# Autodesk Inventor assembly: front
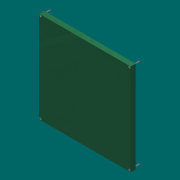
[picture p0: Inventor's stored thumbnail of the model, 180x180]
Saved by Autodesk Inventor 2016 (Build 200138000, 138)
## iProperties
Created: 2015-10-19
Part Number: front
Document SubType Name: Assembly
Designer: Sawaiz
Author: Sawaiz
## Documents named in this file (4)
- C:\Users\Sawaiz\OneDrive\projects\modularRICH\frame\front.iam
- C:\Users\Sawaiz\OneDrive\projects\modularRICH\frame\front.ipt
- C:\Users\Sawaiz\OneDrive\projects\modularRICH\frame\frontBackORing.ipt
- C:\Users\Sawaiz\OneDrive\projects\modularRICH\frame\0x0.5flatPhilips.ipt
## Components (6 placed, 3 different names)
1. front:1 — Mate:1, Mate:2, Mate:3, Mate:4, Flush:1, Mate:5, Mate:6, Mate:7, Flush:2, Flush:3, Flush:4, Flush:5
2. frontBackORing:1 — Mate:1, Mate:2, Mate:3
3. 0x0.5flatPhilips:1 — Mate:4, Flush:1, Flush:5
4. 0x0.5flatPhilips:2 — Mate:5, Flush:4
5. 0x0.5flatPhilips:3 — Mate:6, Flush:3
6. 0x0.5flatPhilips:4 — Mate:7, Flush:2
## Relationships (12: Mate 7, Flush 5)
- Mate:1: front:1 ↔ frontBackORing:1
- Mate:2: front:1 ↔ frontBackORing:1
- Mate:3: front:1 ↔ frontBackORing:1
- Mate:4: front:1 ↔ 0x0.5flatPhilips:1
- Flush:1: front:1 ↔ 0x0.5flatPhilips:1
- Mate:5: front:1 ↔ 0x0.5flatPhilips:2
- Mate:6: front:1 ↔ 0x0.5flatPhilips:3
- Mate:7: front:1 ↔ 0x0.5flatPhilips:4
- Flush:2: front:1 ↔ 0x0.5flatPhilips:4
- Flush:3: front:1 ↔ 0x0.5flatPhilips:3
- Flush:4: front:1 ↔ 0x0.5flatPhilips:2
- Flush:5: front:1 ↔ 0x0.5flatPhilips:1
